# Autodesk Inventor assembly: CompleteCam
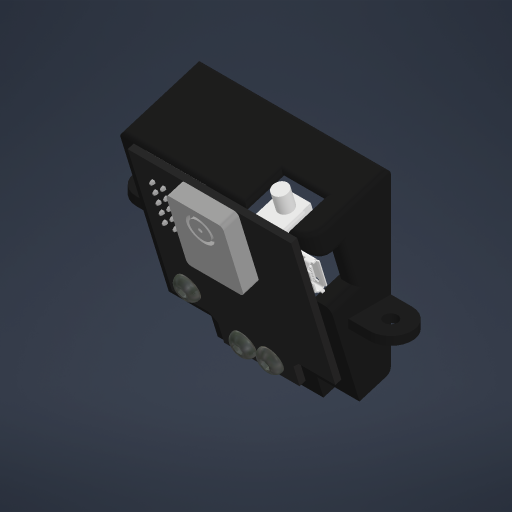
[picture p0: Inventor's stored thumbnail of the model, 512x512]
Saved by Autodesk Inventor 2023 (Build 270158000, 158)
## iProperties
Created: 2023-03-06
Part Number: CompleteCam
Document SubType Name: Assembly
Designer: Elias Braun
Author: Elias Braun
## Documents named in this file (6)
- C:\Users\Elias Braun\Nextcloud2\RoboCup2023\Cam\CompleteCam.iam
- C:\Users\Elias Braun\Nextcloud2\RoboCup2023\Cam\Pixy2-Bracket.ipt
- C:\Users\Elias Braun\Nextcloud2\RoboCup2023\Cam\Pixy2\pixy2Pixy 2.iam
- C:\Users\Elias Braun\Documents\Inventor\Content Center Files\R2023\en-US\ISO 7380-1\ISO 7380-1 - M3 x 12.ipt
- C:\Users\Elias Braun\Documents\Inventor\Content Center Files\R2023\en-US\ISO 7380-1\ISO 7380-1 - M3 x 16.ipt
- C:\Users\Elias Braun\Documents\Inventor\Content Center Files\R2023\en-US\ISO 4035(2)\ISO 4035 - M3 - ISO.ipt
## Components (8 placed, 5 different names)
1. Pixy2-Bracket:1 — Mate:1, Mate:2, Mate:3, Mate:4, Mate:5, Mate:6, Mate:9
2. pixy2Pixy 2:1 [sub-assembly] — Mate:1, Mate:2, Mate:3, Mate:4, Mate:7, Mate:8, Mate:10
3. ISO 7380-1 M3 x 16:1 — Mate:9, Mate:10, Mate:13
4. ISO 7380-1 M3 x 12:2 — Mate:6, Mate:8, Mate:11, Mate:14
5. ISO 7380-1 M3 x 12:1 — Mate:5, Mate:7, Mate:12
6. ISO 4035 M3:3 — Mate:11, Mate:14
7. ISO 4035 M3:2 — Mate:12
8. ISO 4035 M3:1 — Mate:13
## Relationships (14: Mate 14)
- Mate:1: Pixy2-Bracket:1 ↔ pixy2Pixy 2:1
- Mate:2: Pixy2-Bracket:1 ↔ pixy2Pixy 2:1
- Mate:3: Pixy2-Bracket:1 ↔ pixy2Pixy 2:1
- Mate:4: Pixy2-Bracket:1 ↔ pixy2Pixy 2:1
- Mate:5: Pixy2-Bracket:1 ↔ ISO 7380-1 M3 x 12:1
- Mate:6: Pixy2-Bracket:1 ↔ ISO 7380-1 M3 x 12:2
- Mate:7: pixy2Pixy 2:1 ↔ ISO 7380-1 M3 x 12:1
- Mate:8: pixy2Pixy 2:1 ↔ ISO 7380-1 M3 x 12:2
- Mate:9: Pixy2-Bracket:1 ↔ ISO 7380-1 M3 x 16:1
- Mate:10: pixy2Pixy 2:1 ↔ ISO 7380-1 M3 x 16:1
- Mate:11: ISO 7380-1 M3 x 12:2 ↔ ISO 4035 M3:3
- Mate:12: ISO 7380-1 M3 x 12:1 ↔ ISO 4035 M3:2
- Mate:13: ISO 7380-1 M3 x 16:1 ↔ ISO 4035 M3:1
- Mate:14: ISO 7380-1 M3 x 12:2 ↔ ISO 4035 M3:3
